# Autodesk Inventor assembly: 기본틀
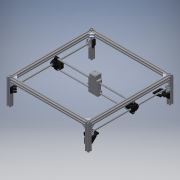
[picture p0: Inventor's stored thumbnail of the model, 180x180]
Saved by Autodesk Inventor 2018 (Build 220112000, 112)
## iProperties
Created: 2019-01-19
Part Number: 기본틀
Document SubType Name: Assembly
Designer: User
Author: User
## Documents named in this file (18)
- C:\Users\User\3D Objects\기본틀.iam
- C:\Users\User\3D Objects\470mm 2020.ipt
- C:\Users\User\3D Objects\150mm 2020.ipt
- C:\Users\User\3D Objects\shf8\SHF8.ipt
- C:\Users\User\3D Objects\600mm 2020.ipt
- C:\Users\User\3D Objects\연마봉 8pi 470mm.ipt
- C:\Users\User\3D Objects\corner bracket\RS-CCB-2017-5 [Cast Aluminum Corner Bracket].ipt
- C:\Users\User\3D Objects\lmuu\lm8uu.iam
- C:\Users\User\3D Objects\lmuu\XY_Clamp_v1.1.ipt
- C:\Users\User\3D Objects\lmuu\XY_Joiner_v1.1.ipt
- C:\Users\User\3D Objects\lmuu\XY_Idler.ipt
- C:\Users\User\3D Objects\lmuu\XY_Motor_left.ipt
- C:\Users\User\3D Objects\lmuu\XY_Motor_right.ipt
- C:\Users\User\3D Objects\lmuu\전자석.ipt
- C:\Users\User\3D Objects\x 캐리지.ipt
- C:\Users\User\3D Objects\x 캐리지 덮개.ipt
- C:\Users\User\3D Objects\x 캐리지 벨트고정.ipt
- C:\Users\User\3D Objects\lmuu\Y_EndStop.ipt
## Components (47 placed, 18 different names)
1. y축 450mm:1 — 메이트:2, 플러쉬:3, 플러쉬:4, 메이트:7, 플러쉬:13, 플러쉬:14, 메이트:18, 메이트:20, 메이트:68, 메이트:74
2. x축 470mm:1 — 메이트:1, 플러쉬:1, 플러쉬:2, 메이트:3, 플러쉬:5, 플러쉬:6, 메이트:15, 플러쉬:25, 메이트:17, 플러쉬:26, 메이트:30, 메이트:73
3. x축 470mm:2 — 메이트:6, 플러쉬:11, 플러쉬:12, 메이트:8, 플러쉬:15, 플러쉬:16, 메이트:19, 플러쉬:27, 메이트:22, 메이트:33, 플러쉬:47, 메이트:70
4. 150mm 2020:1 — 메이트:1, 플러쉬:1, 플러쉬:2, 메이트:2, 플러쉬:3, 플러쉬:4, 메이트:23, 플러쉬:29, 메이트:48, 접선:9, 접선:10, 메이트:72, 플러쉬:53, 메이트:75, 플러쉬:54
5. 150mm 2020:2 — 메이트:3, 플러쉬:5, 플러쉬:6, 메이트:10, 플러쉬:18, 플러쉬:19, 플러쉬:30, 메이트:24, 메이트:28, 플러쉬:37, 메이트:31, 메이트:47, 접선:7, 접선:8
6. 150mm 2020:3 — 메이트:6, 플러쉬:11, 플러쉬:12, 메이트:11, 플러쉬:20, 플러쉬:21, 메이트:25, 플러쉬:31, 메이트:34, 메이트:36, 플러쉬:38, 메이트:49, 메이트:50
7. 150mm 2020:4 — 메이트:7, 플러쉬:13, 플러쉬:14, 메이트:8, 플러쉬:15, 플러쉬:16, 메이트:26, 플러쉬:32, 메이트:51, 메이트:52, 메이트:69, 플러쉬:51, 메이트:71, 플러쉬:52
8. SHF8:1 — 메이트:26, 플러쉬:32, 접선:3, 플러쉬:35, 접선:12
9. 450mm 2020:2 — 메이트:10, 플러쉬:18, 플러쉬:19, 메이트:11, 플러쉬:20, 플러쉬:21, 메이트:16, 메이트:21, 플러쉬:28, 메이트:29, 메이트:37
10. SHF8:2 — 메이트:23, 플러쉬:29, 접선:2, 플러쉬:34
11. SHF8:3 — 메이트:25, 플러쉬:31, 접선:4, 플러쉬:36, 접선:6, 접선:11
12. RS-CCB-2017-5 [Cast Aluminum Corner Bracket]:1 — 메이트:15, 플러쉬:25, 메이트:16
13. RS-CCB-2017-5 [Cast Aluminum Corner Bracket]:2 — 메이트:17, 플러쉬:26, 메이트:18
14. RS-CCB-2017-5 [Cast Aluminum Corner Bracket]:3 — 메이트:19, 플러쉬:27, 메이트:20
15. RS-CCB-2017-5 [Cast Aluminum Corner Bracket]:4 — 메이트:21, 플러쉬:28, 메이트:22
16. SHF8:4 — 플러쉬:30, 메이트:24, 접선:1, 플러쉬:33, 접선:5
17. 연마봉 8pi 470mm:5 — 접선:1, 플러쉬:33, 접선:2, 플러쉬:34, 메이트:38
18. 연마봉 8pi 470mm:6 — 접선:3, 플러쉬:35, 접선:4, 플러쉬:36, 메이트:39
19. RS-CCB-2017-5 [Cast Aluminum Corner Bracket]:5 — 메이트:28, 메이트:29, 플러쉬:37
20. RS-CCB-2017-5 [Cast Aluminum Corner Bracket]:6 — 메이트:30, 메이트:31, 접선:5
21. RS-CCB-2017-5 [Cast Aluminum Corner Bracket]:7 — 메이트:33, 메이트:34, 접선:6, 플러쉬:47
22. RS-CCB-2017-5 [Cast Aluminum Corner Bracket]:8 — 메이트:36, 메이트:37, 플러쉬:38
23. lm8uu:1 [sub-assembly] — 메이트:38, 메이트:40, 플러쉬:39
24. lm8uu:2 [sub-assembly] — 메이트:39, 메이트:42, 플러쉬:42
25. XY_Clamp_v1.1:1 — 메이트:41, 플러쉬:40, 플러쉬:41
26. XY_Joiner_v1.1:1 — 메이트:40, 플러쉬:39, 메이트:41, 플러쉬:40, 플러쉬:41, 메이트:44, 플러쉬:45, 메이트:46, 플러쉬:46
27. XY_Joiner_v1.1:2 — 메이트:42, 플러쉬:42, 메이트:43, 플러쉬:43, 플러쉬:44, 메이트:45
28. XY_Clamp_v1.1:2 — 메이트:43, 플러쉬:43, 플러쉬:44
29. 연마봉 8pi 470mm:7 — 메이트:44, 플러쉬:45, 메이트:45, 메이트:53, 메이트:55
30. 연마봉 8pi 470mm:8 — 메이트:46, 플러쉬:46, 메이트:54, 메이트:56
31. XY_Idler:1 — 메이트:47, 접선:7, 접선:8
32. XY_Idler:2 — 메이트:48, 접선:9, 접선:10
33. XY_Motor_left:1 — 메이트:49, 메이트:50, 접선:11
34. XY_Motor_right:1 — 메이트:51, 메이트:52, 접선:12
35. lm8uu:3 [sub-assembly] — 메이트:53, 메이트:58, 메이트:63
36. lm8uu:4 [sub-assembly] — 메이트:54, 메이트:60, 메이트:61
37. lm8uu:5 [sub-assembly] — 메이트:55, 메이트:59
38. lm8uu:6 [sub-assembly] — 메이트:56, 메이트:62
39. 전자석:1 — 메이트:64, 접선:13
40. x 캐리지:1 — 메이트:58, 메이트:59, 메이트:60, 메이트:61, 메이트:62, 메이트:63, 메이트:64, 접선:13, 메이트:65, 플러쉬:48, 플러쉬:49, 메이트:66, 플러쉬:50
41. x 캐리지 덮개:1 — 메이트:65, 플러쉬:48, 플러쉬:49, 메이트:67
42. x 캐리지 벨트고정:1 — 메이트:66, 메이트:67, 플러쉬:50
43. Y_EndStop:1
44. RS-CCB-2017-5 [Cast Aluminum Corner Bracket]:9 — 메이트:68, 메이트:69, 플러쉬:51
45. RS-CCB-2017-5 [Cast Aluminum Corner Bracket]:10 — 메이트:70, 메이트:71, 플러쉬:52
46. RS-CCB-2017-5 [Cast Aluminum Corner Bracket]:11 — 메이트:72, 메이트:73, 플러쉬:53
47. RS-CCB-2017-5 [Cast Aluminum Corner Bracket]:12 — 메이트:74, 메이트:75, 플러쉬:54
## Relationships (124: Mate 65, Flush 46, Tangent 13)
- 메이트:1 [Mate]: x축 470mm:1 ↔ 150mm 2020:1
- 플러쉬:1 [Flush]: x축 470mm:1 ↔ 150mm 2020:1
- 플러쉬:2 [Flush]: x축 470mm:1 ↔ 150mm 2020:1
- 메이트:2 [Mate]: y축 450mm:1 ↔ 150mm 2020:1
- 플러쉬:3 [Flush]: y축 450mm:1 ↔ 150mm 2020:1
- 플러쉬:4 [Flush]: y축 450mm:1 ↔ 150mm 2020:1
- 메이트:3 [Mate]: x축 470mm:1 ↔ 150mm 2020:2
- 플러쉬:5 [Flush]: x축 470mm:1 ↔ 150mm 2020:2
- 플러쉬:6 [Flush]: x축 470mm:1 ↔ 150mm 2020:2
- 메이트:6 [Mate]: x축 470mm:2 ↔ 150mm 2020:3
- 플러쉬:11 [Flush]: x축 470mm:2 ↔ 150mm 2020:3
- 플러쉬:12 [Flush]: x축 470mm:2 ↔ 150mm 2020:3
- 메이트:7 [Mate]: y축 450mm:1 ↔ 150mm 2020:4
- 플러쉬:13 [Flush]: y축 450mm:1 ↔ 150mm 2020:4
- 플러쉬:14 [Flush]: y축 450mm:1 ↔ 150mm 2020:4
- 메이트:8 [Mate]: x축 470mm:2 ↔ 150mm 2020:4
- 플러쉬:15 [Flush]: x축 470mm:2 ↔ 150mm 2020:4
- 플러쉬:16 [Flush]: x축 470mm:2 ↔ 150mm 2020:4
- 메이트:10 [Mate]: 150mm 2020:2 ↔ 450mm 2020:2
- 플러쉬:18 [Flush]: 150mm 2020:2 ↔ 450mm 2020:2
- 플러쉬:19 [Flush]: 150mm 2020:2 ↔ 450mm 2020:2
- 메이트:11 [Mate]: 150mm 2020:3 ↔ 450mm 2020:2
- 플러쉬:20 [Flush]: 150mm 2020:3 ↔ 450mm 2020:2
- 플러쉬:21 [Flush]: 150mm 2020:3 ↔ 450mm 2020:2
- 메이트:15 [Mate]: x축 470mm:1 ↔ RS-CCB-2017-5 [Cast Aluminum Corner Bracket]:1
- 플러쉬:25 [Flush]: x축 470mm:1 ↔ RS-CCB-2017-5 [Cast Aluminum Corner Bracket]:1
- 메이트:16 [Mate]: 450mm 2020:2 ↔ RS-CCB-2017-5 [Cast Aluminum Corner Bracket]:1
- 메이트:17 [Mate]: x축 470mm:1 ↔ RS-CCB-2017-5 [Cast Aluminum Corner Bracket]:2
- 플러쉬:26 [Flush]: x축 470mm:1 ↔ RS-CCB-2017-5 [Cast Aluminum Corner Bracket]:2
- 메이트:18 [Mate]: y축 450mm:1 ↔ RS-CCB-2017-5 [Cast Aluminum Corner Bracket]:2
- 메이트:19 [Mate]: x축 470mm:2 ↔ RS-CCB-2017-5 [Cast Aluminum Corner Bracket]:3
- 플러쉬:27 [Flush]: x축 470mm:2 ↔ RS-CCB-2017-5 [Cast Aluminum Corner Bracket]:3
- 메이트:20 [Mate]: y축 450mm:1 ↔ RS-CCB-2017-5 [Cast Aluminum Corner Bracket]:3
- 메이트:21 [Mate]: 450mm 2020:2 ↔ RS-CCB-2017-5 [Cast Aluminum Corner Bracket]:4
- 플러쉬:28 [Flush]: 450mm 2020:2 ↔ RS-CCB-2017-5 [Cast Aluminum Corner Bracket]:4
- 메이트:22 [Mate]: x축 470mm:2 ↔ RS-CCB-2017-5 [Cast Aluminum Corner Bracket]:4
- 메이트:23 [Mate]: 150mm 2020:1 ↔ SHF8:2
- 플러쉬:29 [Flush]: 150mm 2020:1 ↔ SHF8:2
- 플러쉬:30 [Flush]: 150mm 2020:2 ↔ SHF8:4
- 메이트:24 [Mate]: 150mm 2020:2 ↔ SHF8:4
- 메이트:25 [Mate]: 150mm 2020:3 ↔ SHF8:3
- 플러쉬:31 [Flush]: 150mm 2020:3 ↔ SHF8:3
- 메이트:26 [Mate]: 150mm 2020:4 ↔ SHF8:1
- 플러쉬:32 [Flush]: 150mm 2020:4 ↔ SHF8:1
- 접선:1 [Tangent]: SHF8:4 ↔ 연마봉 8pi 470mm:5
- 플러쉬:33 [Flush]: SHF8:4 ↔ 연마봉 8pi 470mm:5
- 접선:2 [Tangent]: SHF8:2 ↔ 연마봉 8pi 470mm:5
- 플러쉬:34 [Flush]: SHF8:2 ↔ 연마봉 8pi 470mm:5
- 접선:3 [Tangent]: SHF8:1 ↔ 연마봉 8pi 470mm:6
- 플러쉬:35 [Flush]: SHF8:1 ↔ 연마봉 8pi 470mm:6
- 접선:4 [Tangent]: SHF8:3 ↔ 연마봉 8pi 470mm:6
- 플러쉬:36 [Flush]: SHF8:3 ↔ 연마봉 8pi 470mm:6
- 메이트:28 [Mate]: 150mm 2020:2 ↔ RS-CCB-2017-5 [Cast Aluminum Corner Bracket]:5
- 메이트:29 [Mate]: 450mm 2020:2 ↔ RS-CCB-2017-5 [Cast Aluminum Corner Bracket]:5
- 플러쉬:37 [Flush]: 150mm 2020:2 ↔ RS-CCB-2017-5 [Cast Aluminum Corner Bracket]:5
- 메이트:30 [Mate]: x축 470mm:1 ↔ RS-CCB-2017-5 [Cast Aluminum Corner Bracket]:6
- 메이트:31 [Mate]: 150mm 2020:2 ↔ RS-CCB-2017-5 [Cast Aluminum Corner Bracket]:6
- 메이트:33 [Mate]: x축 470mm:2 ↔ RS-CCB-2017-5 [Cast Aluminum Corner Bracket]:7
- 메이트:34 [Mate]: 150mm 2020:3 ↔ RS-CCB-2017-5 [Cast Aluminum Corner Bracket]:7
- 메이트:36 [Mate]: 150mm 2020:3 ↔ RS-CCB-2017-5 [Cast Aluminum Corner Bracket]:8
- 메이트:37 [Mate]: 450mm 2020:2 ↔ RS-CCB-2017-5 [Cast Aluminum Corner Bracket]:8
- 플러쉬:38 [Flush]: 150mm 2020:3 ↔ RS-CCB-2017-5 [Cast Aluminum Corner Bracket]:8
- 메이트:38 [Mate]: 연마봉 8pi 470mm:5 ↔ lm8uu:1
- 메이트:39 [Mate]: 연마봉 8pi 470mm:6 ↔ lm8uu:2
- 메이트:40 [Mate]: lm8uu:1 ↔ XY_Joiner_v1.1:1
- 플러쉬:39 [Flush]: lm8uu:1 ↔ XY_Joiner_v1.1:1
- 메이트:41 [Mate]: XY_Clamp_v1.1:1 ↔ XY_Joiner_v1.1:1
- 플러쉬:40 [Flush]: XY_Clamp_v1.1:1 ↔ XY_Joiner_v1.1:1
- 플러쉬:41 [Flush]: XY_Clamp_v1.1:1 ↔ XY_Joiner_v1.1:1
- 접선:5 [Tangent]: SHF8:4 ↔ RS-CCB-2017-5 [Cast Aluminum Corner Bracket]:6
- 접선:6 [Tangent]: SHF8:3 ↔ RS-CCB-2017-5 [Cast Aluminum Corner Bracket]:7
- 메이트:42 [Mate]: lm8uu:2 ↔ XY_Joiner_v1.1:2
- 플러쉬:42 [Flush]: lm8uu:2 ↔ XY_Joiner_v1.1:2
- 메이트:43 [Mate]: XY_Joiner_v1.1:2 ↔ XY_Clamp_v1.1:2
- 플러쉬:43 [Flush]: XY_Joiner_v1.1:2 ↔ XY_Clamp_v1.1:2
- 플러쉬:44 [Flush]: XY_Joiner_v1.1:2 ↔ XY_Clamp_v1.1:2
- 메이트:44 [Mate]: XY_Joiner_v1.1:1 ↔ 연마봉 8pi 470mm:7
- 플러쉬:45 [Flush]: XY_Joiner_v1.1:1 ↔ 연마봉 8pi 470mm:7
- 메이트:45 [Mate]: XY_Joiner_v1.1:2 ↔ 연마봉 8pi 470mm:7
- 메이트:46 [Mate]: XY_Joiner_v1.1:1 ↔ 연마봉 8pi 470mm:8
- 플러쉬:46 [Flush]: XY_Joiner_v1.1:1 ↔ 연마봉 8pi 470mm:8
- 메이트:47 [Mate]: 150mm 2020:2 ↔ XY_Idler:1
- 접선:7 [Tangent]: 150mm 2020:2 ↔ XY_Idler:1
- 접선:8 [Tangent]: 150mm 2020:2 ↔ XY_Idler:1
- 메이트:48 [Mate]: 150mm 2020:1 ↔ XY_Idler:2
- 접선:9 [Tangent]: 150mm 2020:1 ↔ XY_Idler:2
- 접선:10 [Tangent]: 150mm 2020:1 ↔ XY_Idler:2
- 플러쉬:47 [Flush]: x축 470mm:2 ↔ RS-CCB-2017-5 [Cast Aluminum Corner Bracket]:7
- 메이트:49 [Mate]: 150mm 2020:3 ↔ XY_Motor_left:1
- 메이트:50 [Mate]: 150mm 2020:3 ↔ XY_Motor_left:1
- 접선:11 [Tangent]: SHF8:3 ↔ XY_Motor_left:1
- 메이트:51 [Mate]: 150mm 2020:4 ↔ XY_Motor_right:1
- 메이트:52 [Mate]: 150mm 2020:4 ↔ XY_Motor_right:1
- 접선:12 [Tangent]: SHF8:1 ↔ XY_Motor_right:1
- 메이트:53 [Mate]: 연마봉 8pi 470mm:7 ↔ lm8uu:3
- 메이트:54 [Mate]: 연마봉 8pi 470mm:8 ↔ lm8uu:4
- 메이트:55 [Mate]: 연마봉 8pi 470mm:7 ↔ lm8uu:5
- 메이트:56 [Mate]: 연마봉 8pi 470mm:8 ↔ lm8uu:6
- 메이트:58 [Mate]: lm8uu:3 ↔ x 캐리지:1
- 메이트:59 [Mate]: lm8uu:5 ↔ x 캐리지:1
- 메이트:60 [Mate]: lm8uu:4 ↔ x 캐리지:1
- 메이트:61 [Mate]: lm8uu:4 ↔ x 캐리지:1
- 메이트:62 [Mate]: lm8uu:6 ↔ x 캐리지:1
- 메이트:63 [Mate]: lm8uu:3 ↔ x 캐리지:1
- 메이트:64 [Mate]: 전자석:1 ↔ x 캐리지:1
- 접선:13 [Tangent]: 전자석:1 ↔ x 캐리지:1
- 메이트:65 [Mate]: x 캐리지:1 ↔ x 캐리지 덮개:1
- 플러쉬:48 [Flush]: x 캐리지:1 ↔ x 캐리지 덮개:1
- 플러쉬:49 [Flush]: x 캐리지:1 ↔ x 캐리지 덮개:1
- 메이트:66 [Mate]: x 캐리지:1 ↔ x 캐리지 벨트고정:1
- 메이트:67 [Mate]: x 캐리지 덮개:1 ↔ x 캐리지 벨트고정:1
- 플러쉬:50 [Flush]: x 캐리지:1 ↔ x 캐리지 벨트고정:1
- 메이트:68 [Mate]: y축 450mm:1 ↔ RS-CCB-2017-5 [Cast Aluminum Corner Bracket]:9
- 메이트:69 [Mate]: 150mm 2020:4 ↔ RS-CCB-2017-5 [Cast Aluminum Corner Bracket]:9
- 플러쉬:51 [Flush]: 150mm 2020:4 ↔ RS-CCB-2017-5 [Cast Aluminum Corner Bracket]:9
- 메이트:70 [Mate]: x축 470mm:2 ↔ RS-CCB-2017-5 [Cast Aluminum Corner Bracket]:10
- 메이트:71 [Mate]: 150mm 2020:4 ↔ RS-CCB-2017-5 [Cast Aluminum Corner Bracket]:10
- 플러쉬:52 [Flush]: 150mm 2020:4 ↔ RS-CCB-2017-5 [Cast Aluminum Corner Bracket]:10
- 메이트:72 [Mate]: 150mm 2020:1 ↔ RS-CCB-2017-5 [Cast Aluminum Corner Bracket]:11
- 메이트:73 [Mate]: x축 470mm:1 ↔ RS-CCB-2017-5 [Cast Aluminum Corner Bracket]:11
- 플러쉬:53 [Flush]: 150mm 2020:1 ↔ RS-CCB-2017-5 [Cast Aluminum Corner Bracket]:11
- 메이트:74 [Mate]: y축 450mm:1 ↔ RS-CCB-2017-5 [Cast Aluminum Corner Bracket]:12
- 메이트:75 [Mate]: 150mm 2020:1 ↔ RS-CCB-2017-5 [Cast Aluminum Corner Bracket]:12
- 플러쉬:54 [Flush]: 150mm 2020:1 ↔ RS-CCB-2017-5 [Cast Aluminum Corner Bracket]:12
